# Autodesk Inventor assembly: front_rear_unit_assembly
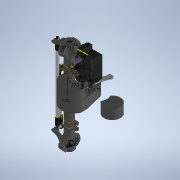
[picture p0: Inventor's stored thumbnail of the model, 180x180]
Saved by Autodesk Inventor 2020 (Build 240168000, 168)
## iProperties
Created: 2019-11-28
Part Number: front_rear_unit_assembly
Document SubType Name: Assembly
Designer: maste
Author: maste
## Documents named in this file (11)
- C:\Users\maste\Documents\GitHub\autobot\robot_model\front_rear_unit_assembly.iam
- C:\Users\maste\Documents\GitHub\autobot\robot_model\RCT-P004_front_rear_axle_simplified.ipt
- C:\Users\maste\Documents\GitHub\autobot\robot_model\RCT-P006_steering_knuckle_OK.ipt
- C:\Users\maste\Documents\GitHub\autobot\robot_model\RCT-P006_steering_knuckle_right_OK.ipt
- C:\Users\maste\Documents\GitHub\autobot\robot_model\RCT-T003_front_rear_steering_linkage_assembly.iam
- C:\Users\maste\Documents\GitHub\autobot\robot_model\RCT-H022_washer_31_60_05.ipt
- C:\Users\maste\Documents\GitHub\autobot\robot_model\H016.ipt
- C:\Users\maste\Documents\GitHub\autobot\robot_model\RCT-T004_front_rear_servo_linkage_assembly.iam
- C:\Users\maste\Documents\GitHub\autobot\robot_model\servo_plate_assembly.iam
- C:\Users\maste\Documents\GitHub\autobot\robot_model\servo_link_assembly.iam
- C:\Users\maste\Documents\GitHub\autobot\robot_model\RCT-H111_upper_link_mount.ipt
## Components (13 placed, 10 different names)
1. RCT-P004_front_rear_axle_simplified:1 — Mate:1, Mate:2, Flush:1, Mate:18, Mate:19, Flush:2, Mate:20, Mate:21, Mate:22
2. RCT-P006_steering_knuckle_OK:1 — Mate:1, Mate:5, Mate:6, Mate:9, Mate:18
3. RCT-P006_steering_knuckle_right_OK:1 — Mate:2, Mate:3, Mate:4, Mate:7, Mate:17, Mate:19
4. RCT-T003_front_rear_steering_linkage_assembly:1 [sub-assembly] — Ball:1, Ball:2
5. RCT-H022_washer_31_60_05:1 — Mate:3, Mate:4, Mate:8
6. RCT-H022_washer_31_60_05:2 — Mate:5, Mate:6, Mate:10
7. H016:1 — Mate:7, Mate:8, Mate:11, Mate:12, Ball:1
8. H016:2 — Mate:9, Mate:10, Ball:2
9. H016:3 — Mate:11, Mate:12, Ball:3
10. RCT-T004_front_rear_servo_linkage_assembly:1 [sub-assembly] — Ball:3, Ball:4
11. servo_plate_assembly:1 [sub-assembly] — Mate:13, Mate:14, Mate:17, Flush:1, Flush:2
12. servo_link_assembly:1 [sub-assembly] — Mate:13, Mate:14, Ball:4
13. RCT-H111_upper_link_mount:1 — Mate:20, Mate:21, Mate:22
## Relationships (26: Mate 20, BallJoint 4, Flush 2)
- Mate:1: RCT-P004_front_rear_axle_simplified:1 ↔ RCT-P006_steering_knuckle_OK:1
- Mate:2: RCT-P004_front_rear_axle_simplified:1 ↔ RCT-P006_steering_knuckle_right_OK:1
- Mate:3: RCT-P006_steering_knuckle_right_OK:1 ↔ RCT-H022_washer_31_60_05:1
- Mate:4: RCT-P006_steering_knuckle_right_OK:1 ↔ RCT-H022_washer_31_60_05:1
- Mate:5: RCT-P006_steering_knuckle_OK:1 ↔ RCT-H022_washer_31_60_05:2
- Mate:6: RCT-P006_steering_knuckle_OK:1 ↔ RCT-H022_washer_31_60_05:2
- Mate:7: RCT-P006_steering_knuckle_right_OK:1 ↔ H016:1
- Mate:8: RCT-H022_washer_31_60_05:1 ↔ H016:1
- Mate:9: RCT-P006_steering_knuckle_OK:1 ↔ H016:2
- Mate:10: RCT-H022_washer_31_60_05:2 ↔ H016:2
- Mate:11: H016:1 ↔ H016:3
- Mate:12: H016:1 ↔ H016:3
- Ball:1: RCT-T003_front_rear_steering_linkage_assembly:1 ↔ H016:1
- Ball:2: RCT-T003_front_rear_steering_linkage_assembly:1 ↔ H016:2
- Ball:3: H016:3 ↔ RCT-T004_front_rear_servo_linkage_assembly:1
- Mate:13: servo_plate_assembly:1 ↔ servo_link_assembly:1
- Mate:14: servo_plate_assembly:1 ↔ servo_link_assembly:1
- Mate:17 (9 mm): RCT-P006_steering_knuckle_right_OK:1 ↔ servo_plate_assembly:1
- Flush:1: RCT-P004_front_rear_axle_simplified:1 ↔ servo_plate_assembly:1
- Ball:4: RCT-T004_front_rear_servo_linkage_assembly:1 ↔ servo_link_assembly:1
- Mate:18 (1 mm): RCT-P004_front_rear_axle_simplified:1 ↔ RCT-P006_steering_knuckle_OK:1
- Mate:19 (1 mm): RCT-P004_front_rear_axle_simplified:1 ↔ RCT-P006_steering_knuckle_right_OK:1
- Flush:2 (-12 mm): RCT-P004_front_rear_axle_simplified:1 ↔ servo_plate_assembly:1
- Mate:20: RCT-P004_front_rear_axle_simplified:1 ↔ RCT-H111_upper_link_mount:1
- Mate:21: RCT-P004_front_rear_axle_simplified:1 ↔ RCT-H111_upper_link_mount:1
- Mate:22: RCT-P004_front_rear_axle_simplified:1 ↔ RCT-H111_upper_link_mount:1
